# Autodesk Inventor assembly: linkageAssembly
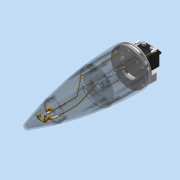
[picture p0: Inventor's stored thumbnail of the model, 180x180]
Saved by Autodesk Inventor 2017 (Build 210142000, 142)
## iProperties
Created: 2016-12-11
Part Number: linkageAssembly
Document SubType Name: Assembly
Designer: techn
Author: techn
## Documents named in this file (18)
- D:\OneDrive\Documents\Other Projects\Submarine\CAD\aft\linkageAssembly.iam
- D:\OneDrive\Documents\Other Projects\Submarine\CAD\aft\AftSectionAirtightRear.ipt
- D:\OneDrive\Documents\Other Projects\Submarine\CAD\aft\AftSectionWithSteeringLinkages.ipt
- D:\OneDrive\Documents\Other Projects\Submarine\CAD\aft\RearmostAftSection.ipt
- D:\OneDrive\Documents\Other Projects\Submarine\CAD\common\steeringYoke3mmShaft.ipt
- D:\OneDrive\Documents\Other Projects\Submarine\CAD\aft\aftSectionAirtightCap.ipt
- D:\OneDrive\Documents\Other Projects\Submarine\CAD\common\AluminumSealingDisc.ipt
- D:\OneDrive\Documents\Other Projects\Submarine\CAD\midships\AftServoSection\rearServoAttachmentPlate.ipt
- D:\OneDrive\Documents\Other Projects\Submarine\CAD\common\HitecServo\HitecServoAssembly.iam
- D:\OneDrive\Documents\Other Projects\Submarine\CAD\common\HitecServo\ServoHorn10mmPitch.ipt
- D:\OneDrive\Documents\Other Projects\Submarine\CAD\aft\planeLinkages\2mmBentFromSealDive.ipt
- D:\OneDrive\Documents\Other Projects\Submarine\CAD\aft\planeLinkages\2mmToDive.ipt
- D:\OneDrive\Documents\Other Projects\Submarine\CAD\aft\planeLinkages\2mmToSeal.ipt
- D:\OneDrive\Documents\Other Projects\Submarine\CAD\aft\planeLinkages\2mmToServo.ipt
- D:\OneDrive\Documents\Other Projects\Submarine\CAD\aft\planeLinkages\3mmHollowExpander.ipt
- D:\OneDrive\Documents\Other Projects\Submarine\CAD\aft\planeLinkages\metalClevisis.ipt
- D:\OneDrive\Documents\Other Projects\Submarine\CAD\aft\planeLinkages\2mmBentFromSealRudder.ipt
- D:\OneDrive\Documents\Other Projects\Submarine\CAD\aft\planeLinkages\2mmToRudder.ipt
## Components (26 placed, 17 different names)
1. AftSectionAirtightRear:1 — Mate:1, Mate:2, Mate:5, Mate:6, Mate:7, Mate:45, Mate:46
2. AftSectionWithSteeringLinkages:1 — Mate:1, Mate:2, Mate:30, Mate:31
3. AluminumSealingDisc:1 — Mate:8, Mate:9, Mate:10, Mate:11, Mate:12, Mate:13
4. rearServoAttachmentPlate:1 — Mate:11, Mate:12, Mate:13, Mate:14, Mate:15, Mate:16, Mate:17, Mate:18, Mate:19
5. HitecServoAssembly:1 [sub-assembly] — Mate:14, Mate:15, Mate:16, Mate:20, Mate:23, Angle:3
6. HitecServoAssembly:2 [sub-assembly] — Mate:17, Mate:18, Mate:19, Mate:21, Mate:22, Angle:4
7. ServoHorn10mmPitch:1 — Mate:20, Mate:23, Angle:3, Mate:37
8. ServoHorn10mmPitch:2 — Mate:21, Mate:22, Angle:4, Mate:36
9. aftSectionAirtightCap:2 — Mate:5, Mate:6, Mate:7, Mate:8, Mate:9, Mate:10
10. RearmostAftSection:2 — Mate:28, Mate:29, Mate:30, Mate:31
11. steeringYoke3mmShaft:3 — Mate:29, Mate:59, Mate:60
12. steeringYoke3mmShaft:4 — Mate:28, Mate:61, Mate:77
13. metalClevisis:5 — Mate:36, Mate:71, Mate:72
14. metalClevisis:6 — Mate:37, Mate:55, Mate:56
15. 2mmToServo:7 — Mate:55, Mate:56, Ball:3
16. 2mmToSeal:4 — Mate:47, Mate:49, Ball:2
17. 2mmToSeal:5 — Mate:48, Mate:50, Ball:3
18. 3mmHollowExpander:4 — Mate:46, Mate:48, Mate:50, Mate:73, Mate:74
19. 3mmHollowExpander:5 — Mate:45, Mate:47, Mate:49, Mate:57, Mate:58
20. 2mmToDive:1 — Mate:57, Mate:58, Ball:1
21. metalClevisis:7 — Mate:59, Mate:60, Mate:69, Mate:70
22. metalClevisis:8 — Mate:61, Mate:75, Mate:76, Mate:77
23. 2mmBentFromSealDive:2 — Ball:1, Mate:69, Mate:70
24. 2mmToServo:8 — Ball:2, Mate:71, Mate:72
25. 2mmToRudder:1 — Mate:73, Mate:74, Ball:4
26. 2mmBentFromSealRudder:2 — Ball:4, Mate:75, Mate:76
## Relationships (57: Mate 51, BallJoint 4, Angle 2)
- Mate:1: AftSectionAirtightRear:1 ↔ AftSectionWithSteeringLinkages:1
- Mate:2: AftSectionAirtightRear:1 ↔ AftSectionWithSteeringLinkages:1
- Mate:5: AftSectionAirtightRear:1 ↔ aftSectionAirtightCap:2
- Mate:6: AftSectionAirtightRear:1 ↔ aftSectionAirtightCap:2
- Mate:7: AftSectionAirtightRear:1 ↔ aftSectionAirtightCap:2
- Mate:8: AluminumSealingDisc:1 ↔ aftSectionAirtightCap:2
- Mate:9: AluminumSealingDisc:1 ↔ aftSectionAirtightCap:2
- Mate:10: AluminumSealingDisc:1 ↔ aftSectionAirtightCap:2
- Mate:11: AluminumSealingDisc:1 ↔ rearServoAttachmentPlate:1
- Mate:12: AluminumSealingDisc:1 ↔ rearServoAttachmentPlate:1
- Mate:13: AluminumSealingDisc:1 ↔ rearServoAttachmentPlate:1
- Mate:14: rearServoAttachmentPlate:1 ↔ HitecServoAssembly:1
- Mate:15: rearServoAttachmentPlate:1 ↔ HitecServoAssembly:1
- Mate:16: rearServoAttachmentPlate:1 ↔ HitecServoAssembly:1
- Mate:17: rearServoAttachmentPlate:1 ↔ HitecServoAssembly:2
- Mate:18: rearServoAttachmentPlate:1 ↔ HitecServoAssembly:2
- Mate:19: rearServoAttachmentPlate:1 ↔ HitecServoAssembly:2
- Mate:20: HitecServoAssembly:1 ↔ ServoHorn10mmPitch:1
- Mate:21: HitecServoAssembly:2 ↔ ServoHorn10mmPitch:2
- Mate:22: HitecServoAssembly:2 ↔ ServoHorn10mmPitch:2
- Mate:23: HitecServoAssembly:1 ↔ ServoHorn10mmPitch:1
- [Mate]: RearmostAftSection:2 ↔ steeringYoke3mmShaft:4
- [Mate]: RearmostAftSection:2 ↔ steeringYoke3mmShaft:3
- Mate:28 (7.747 mm): RearmostAftSection:2 ↔ steeringYoke3mmShaft:4
- Mate:29 (2.8575 mm): RearmostAftSection:2 ↔ steeringYoke3mmShaft:3
- Mate:30: AftSectionWithSteeringLinkages:1 ↔ RearmostAftSection:2
- Mate:31: AftSectionWithSteeringLinkages:1 ↔ RearmostAftSection:2
- Angle:3 (-10.982 deg): HitecServoAssembly:1 ↔ ServoHorn10mmPitch:1
- Angle:4 (10.982 deg): HitecServoAssembly:2 ↔ ServoHorn10mmPitch:2
- Mate:36: ServoHorn10mmPitch:2 ↔ metalClevisis:5
- Mate:37: ServoHorn10mmPitch:1 ↔ metalClevisis:6
- Mate:45: AftSectionAirtightRear:1 ↔ 3mmHollowExpander:5
- Mate:46: AftSectionAirtightRear:1 ↔ 3mmHollowExpander:4
- Mate:47: 2mmToSeal:4 ↔ 3mmHollowExpander:5
- Mate:48: 2mmToSeal:5 ↔ 3mmHollowExpander:4
- Mate:49 (-25.4 mm): 2mmToSeal:4 ↔ 3mmHollowExpander:5
- Mate:50 (-25.4 mm): 2mmToSeal:5 ↔ 3mmHollowExpander:4
- Mate:55: metalClevisis:6 ↔ 2mmToServo:7
- Mate:56: metalClevisis:6 ↔ 2mmToServo:7
- Mate:57: 3mmHollowExpander:5 ↔ 2mmToDive:1
- Mate:58 (-25.4 mm): 3mmHollowExpander:5 ↔ 2mmToDive:1
- Mate:59: steeringYoke3mmShaft:3 ↔ metalClevisis:7
- Mate:60 (0.762 mm): steeringYoke3mmShaft:3 ↔ metalClevisis:7
- Mate:61: steeringYoke3mmShaft:4 ↔ metalClevisis:8
- Ball:1: 2mmToDive:1 ↔ 2mmBentFromSealDive:2
- Mate:69: metalClevisis:7 ↔ 2mmBentFromSealDive:2
- Mate:70: metalClevisis:7 ↔ 2mmBentFromSealDive:2
- Ball:2: 2mmToSeal:4 ↔ 2mmToServo:8
- Mate:71: metalClevisis:5 ↔ 2mmToServo:8
- Mate:72: metalClevisis:5 ↔ 2mmToServo:8
- Ball:3: 2mmToServo:7 ↔ 2mmToSeal:5
- Mate:73: 3mmHollowExpander:4 ↔ 2mmToRudder:1
- Mate:74 (-25.4 mm): 3mmHollowExpander:4 ↔ 2mmToRudder:1
- Ball:4: 2mmToRudder:1 ↔ 2mmBentFromSealRudder:2
- Mate:75: metalClevisis:8 ↔ 2mmBentFromSealRudder:2
- Mate:76: metalClevisis:8 ↔ 2mmBentFromSealRudder:2
- Mate:77 (0.762 mm): steeringYoke3mmShaft:4 ↔ metalClevisis:8
## Named parameters: d30_d28 = 0 mm, d31_d29 = 0 mm
